# Autodesk Inventor assembly: HTPA22S2M100-K-P4
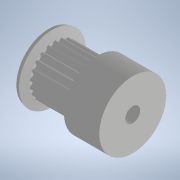
[picture p0: Inventor's stored thumbnail of the model, 180x180]
Saved by Autodesk Inventor 2021 (Build 250183000, 183)
## iProperties
Category: PARTsolutions
Company: MISUMI
Created: 2025-03-04
Part Number: HTPA22S2M100-K-P4
Catalog Web Link: www.cadenas.de
Description: HTPA_ _S2M040, HTPA_ _S2M060, HTPA_ _S2M100, HTPB_ _S2M040, HTPB_ _S2M060, HTPB_ _S2M100, HTPK_ _S2M040, HTPK_ _S2M060, HTPK_ _S2M100, HTPN_ _S2M040, HTPN_ _S2M060, HTPN_ _S2M100, HTPT_ _S2M040, HTPT_ _S2M060, HTPM_ _S2M040, HTPM_ _S2M060, HTPP_ _S2M040, HTPP_ _S2M060, HTPS_ _S2M040, HTPS_ _S2M060, HTPS_ _S2M100-High Torque Timing Pulleys S2M Type
Vendor: MISUMI
Document SubType Name: Assembly
Designer: psAdmin
Manufacturer: MISUMI
Mass: 3.936 g
Surface Area: 24.8143 cm^2
Volume: 3.936 cm^3
Density: 1 g/cm^3
Title: HTPA22S2M100-K-P4
Author: Cadenas PARTsolutions
Comments: High Torque Timing Pulleys S2M Type
PSOL_IDENT_0: {$CADENAS_DATA/23d-libs/misumi/metric/51_timing_pulleys/htpm_s2m_asmtab.prj},744 {VTYP=3D},{STYP=ASS
PSOL_IDENT_1: TAB},{NB=HTPA22S2M100-K-P4},{LINA=HTPA22S2M100-K-P4},{NN=HTPA_ _S2M040, HTPA_ _S2M060, HTPA_ _S2M100
PSOL_IDENT_2: , HTPB_ _S2M040, HTPB_ _S2M060, HTPB_ _S2M100, HTPK_ _S2M040, HTPK_ _S2M060, HTPK_ _S2M100, HTPN_ _S
PSOL_IDENT_3: 2M040, HTPN_ _S2M060, HTPN_ _S2M100, HTPT_ _S2M040, HTPT_ _S2M060, HTPM_ _S2M040, HTPM_ _S2M060, HTP
PSOL_IDENT_4: P_ _S2M040, HTPP_ _S2M060, HTPS_ _S2M040, HTPS_ _S2M060, HTPS_ _S2M100},{DATE=13.01.2023 00:39:47},{
PSOL_IDENT_5: GEOMDATE=09.12.2022 07:33:44},{VERSION=},{LINEID=70},{WBVAR=MATP,ST,TNW,PS,SBS,DD,Z,J,Q,R,S,T,ALT1,A
PSOL_IDENT_6: LT2,M,QSC,QFC,QTC,ALT3,K,KSC,KFC,KTC,ALT4,ZM,ZSC,ZFC,ZTC,ALT5,ALT6,ALT7,FC,ALT8,SRG,ALT9,BTC,TL,ALT1
PSOL_IDENT_7: 0,TPC,ALT11,BC,ALT12,SLH,ALT13,BN},{WBNUMERIC=DD,Z,J,Q,R,S,T,QSC,QFC,QTC,K,KSC,KFC,KTC,ZSC,ZFC,ZTC,F
PSOL_IDENT_8: C,SRG,BTC,TL,BC,SLH,BN}  {NB=HTPA22S2M100-K-P4},{LINA=HTPA22S2M100-K-P4},{KT=DUMMY},{PN=HTPA22S2M100
PSOL_IDENT_9: -K-P4},{TYPE=HTPA},{MATP=A2017},{MATPALG= 'A2017','Aluminum Alloy 2000 series','S45CE','1045 Carbon
PSOL_IDENT_10: Steel Equivalent','SUS304','304 Stainless Steel' },{ST=CA},{STALG= 'CA' , 'Clear Anodize', 'BA','Bla
PSOL_IDENT_11: ck Anodize','HAT','Hard Clear Anodize' , 'ENP' , 'Electroless Nickel Plating' },{NT=22},{TNW=S2M100}
PSOL_IDENT_12: ,{TNWALG= 'S2M040', 'S2M060','S2M100' },{BW=10},{PS=K},{PSALG='A','K'},{SBS=P},{SBSALG='H','Round Ho
PSOL_IDENT_13: le','P','Round Hole + Tap'},{SHSA= 'H', 'Round Hole','V','Stepped Hole','Y','Both Ends Stepped Hole'
PSOL_IDENT_14: ,'WB','Double Stepped Hole' },{SHSB='H','Round Hole','P','Round Hole + Tap','N','New JIS Keywayed Bo
PSOL_IDENT_15: re + Tap (Standard)','NK','New JIS Keywayed Bore + Tap (width 4.0mm, height 1.8mm)','C','Old JIS Key
PSOL_IDENT_16: wayed Bore + Tap','V','Stepped Hole','F','Stepped Hole (Counterbore holes on the boss side)' },{SHSK='
PSOL_IDENT_17: H','Round Hole','P','Round Hole + Tap'},{SBSPN=-P4},{DD=4.00},{DDALG=[3:4/1],4.5,[5:6/1]},{DDHA=[3:4
PSOL_IDENT_18: /1],4.5,[5:6/1],6.35,[7:7/1]},{DDHBK=[3:4/1],4.5,[5:6/1]},{DDPA=0},{DDPBK=[3:4/1],4.5,[5:6/1]},{DDNA=
PSOL_IDENT_19: 0},{DDNBK=0},{DDNK=0},{DDCA=0},{DDCBK=0},{DDVA=0},{DDVF=[3:4/1]},{DDY=[3:5/1]},{DDWB=[3:3/1]},{Z=0},
PSOL_IDENT_20: {ZALG=[0]},{ZQRMIN=6},{ZAMAX=0},{ZBMAX=6},{DDZ=4},{J=0.0},{JALG=[0]},{JMAX=0},{JMIN=2},{JPN=},{QRMAX=
PSOL_IDENT_21: 7},{QRMIN=6},{WBRMAX=-2.00},{WBQMIN=8},{Q=0},{QALG=[0]},{QPN=},{R=0},{RALG=[0]},{S=0.0},{SALG=[0]},{
PSOL_IDENT_22: SPN=},{SMAX=9},{T=0.0},{TALG=[0]},{TPN=},{TMAX=12},{A=11},{W=15},{L=23},{PD=14.01},{OD=13.50},{D=18}
PSOL_IDENT_23: ,{DALG=18},{DE=18},{F=18},{E=11},{BBK=0.000},{TTK=0.0},{TT=1},{WL=23.000},{ALT1=},{ALT1ALG= '','w/o
PSOL_IDENT_24: KC90 (Set Screw Angle)','KC90','with KC90 (Set Screw Angle)' },{ANG=120.000},{ALT1PN=},{ALT2=},{ALT2
PSOL_IDENT_25: ALG= '','Not applicable' },{M=N/A},{MALG= 'N/A' },{MFTALG= 'N/A' },{MSALG= 'N/A' },{M3D=0.000},{KDML=
PSOL_IDENT_26: 0},{ML=0},{MUL=0},{PITCH=0},{QSC=0.0},{QSCALG=0},{QFC=0.0},{QFCALG=0},{QTC=0.0},{QTCALG=0},{QPCDMIN=
PSOL_IDENT_27: 0},{QPCDMINALG=0},{QPCDMAX=14},{ALT2PN=},{ALT3=},{ALT3ALG= '','Not applicable' },{K=0.0},{KALG=0},{K
PSOL_IDENT_28: MIN=4},{KFTMAX=0.0},{KSMAX=0.0},{KSC=0.0},{KSCALG=0},{KFC=0.0},{KFCALG=0},{KTC=0.0},{KTCALG=0},{KPCD
PSOL_IDENT_29: MIN=8},{KPCDMINALG=8},{KPCDMAX=0},{KSCMIN=8.0},{KSCMINALG=8},{ALT3PN=},{ALT4=},{ALT4ALG= '','Not app
PSOL_IDENT_30: licable' },{ALT4MIN=14.5},{ALT4MAX=0.5},{ZM=N/A},{ZMALG= 'N/A' },{ZMSALG= 'N/A' },{ZMFTALG= 'N/A' },
PSOL_IDENT_31: {ZMDD1=0.0},{ZMDD2=0.0},{ZMHH=0.0},{ZSC=0.0},{ZSCALG=[0]},{ZFC=0.0},{ZFCALG=[0]},{ZTC=0.0},{ZTCALG=[
PSOL_IDENT_32: 0]},{ZPCDMIN=0},{ZPCDMINALG=0},{ZPCDMAX=7},{ALT4PN=},{ALT5=},{ALT5ALG= '','Flange Attached','NFC','w
PSOL_IDENT_33: ith NFC (Flange not Attached)' },{ALT5PN=},{ALT6=},{ALT6ALG= '','Not applicable' },{ALT6PN=},{ALT7=}
PSOL_IDENT_34: ,{ALT7ALG= '','w/o FC (Flange Cut)','FC','with FC (Flange Cut)' },{FC=0.0},{FCALG=0},{FCMIN=14.5},{F
PSOL_IDENT_35: CMAX=16.0},{ALT7PN=},{ALT8=},{ALT8ALG= '','Not applicable' },{ALT8ALGALG=14},{ALT8DD2=0},{ALT8MM=0},
PSOL_IDENT_36: {ALT8NN=0},{QC=0},{KC=0},{ZC=0},{SRG=0.0},{SRGALG=[0]},{SRGMAX=0},{DD2=0.0},{MM=0.00},{NN=0.00},{ALT
PSOL_IDENT_37: 8PN=},{ALT9ALG= '','Not applicable' },{ALT9=},{BTC9=6},{TL9=1},{BTC=0},{BTCALG=[0]},{TL=0.0},{TLALG=
PSOL_IDENT_38: [0]},{TLMIN=1.000},{TLMAX=-15.500},{BTCL=0},{BTCD=0},{BTCDALG=11.000},{ALT9PN=},{WLBCTL=23},{ALT10=}
PSOL_IDENT_39: ,{ALT10ALG= '','w/o TPC (Tapped Hole Dimension)','TPC','with TPC (Tapped Hole Dimension)' },{TPC=N/A
PSOL_IDENT_40: },{TPCALG= 'N/A' },{TPCM=3},{ALT10PN=},{ALT11=},{ALT11ALG= '','Not applicable' },{BC=0.0},{BCALG=0},
PSOL_IDENT_41: {BCMIN=6},{BCMAX=7.5},{BCPLANE=18},{M1WBC=18},{ALT11PN=},{ALT12=},{ALT12ALG= '','w/o SLH (Set Screw
PSOL_IDENT_42: Length)','SLH','with SLH (Set Screw Length)' },{SLH=0},{SLHALG=[0]},{ALT12PN=},{ALT13=},{ALT13ALG= ''
PSOL_IDENT_43: , 'Not applicable' },{BN=0.0},{BNALG=0},{BNMIN=8.5},{BNMAX=18},{ALT13PN=},{AC=M3x3},{M1=3},{M1L=3},{
PSOL_IDENT_44: TAP=0.000},{KYY=2},{KTT=7},{PLANE=0},{PPATH=htpm_s2m/htpa_s2m_asmtpl.prj}
NB: HTPA22S2M100-K-P4
NN: 0
NT: 22
NBSYN: $PN.
LINA: HTPA22S2M100-K-P4
CATALOG: Misumi
PN: HTPA22S2M100-K-P4
MATP: Aluminum Alloy 2000 series
ST: Clear Anodize
TNW: S2M100
BW: 10
PS: K
SBS: Round Hole + Tap
DD: 4
Z: 0
J: 0
Q: 0
R: 0
S: 0
T: 0
A: 11
W: 15
L: 23
PD: 14.01
OD: 13.5
D: 18
F: 18
E: 11
TT: 1
ALT1: w/o KC90 (Set Screw Angle)
ALT2: Not applicable
M: N/A
QSC: 0
QFC: 0
QTC: 0
ALT3: Not applicable
K: 0
KSC: 0
KFC: 0
KTC: 0
ALT4: Not applicable
ZM: N/A
ZMDD1: 0
ZMDD2: 0
ZMHH: 0
ZSC: 0
ZFC: 0
ZTC: 0
ALT5: Flange Attached
ALT6: Not applicable
ALT7: w/o FC (Flange Cut)
FC: 0
ALT8: Not applicable
SRG: 0
DD2: 0
MM: 0
ALT9: Not applicable
BTC: 0
TL: 0
BTCL: 0
BTCD: 0
ALT10: w/o TPC (Tapped Hole Dimension)
TPC: N/A
ALT11: Not applicable
BC: 0
ALT12: w/o SLH (Set Screw Length)
SLH: 0
ALT13: Not applicable
BN: 0
AC: M3x3
SUPPLIER: MISUMI
ARTICLENO: HTPA22S2M100-K-P4
BOMINFO: HTPA22S2M100-K-P4
CREATOR: CADENAS GmbH
## Documents named in this file (3)
- e:\temp\worker_COMMON_13\temp\tmp_1524_272_tdsmI\format_0\HTPA22S2M100-K-P4.iam
- e:\temp\worker_COMMON_13\temp\tmp_1524_272_tdsmI\format_0\HTPA22S2M100-K-P4_a.ipt
- e:\temp\worker_COMMON_13\temp\tmp_1524_272_tdsmI\format_0\SET-SCREW3-3.ipt
## Components (3 placed, 2 different names)
1. HTPA22S2M100-K-P4_a:1 — to_s1_Z@1 <-> CP_Z@2, to_s2_Z@1 <-> CP_Z@3
2. SET-SCREW3-3:1 — to_s1_Z@1 <-> CP_Z@2
3. SET-SCREW3-3:2 — to_s2_Z@1 <-> CP_Z@3
## Relationships (2: Mate 2)
- to_s1_Z@1 <-> CP_Z@2 [Mate]: HTPA22S2M100-K-P4_a:1 ↔ SET-SCREW3-3:1
- to_s2_Z@1 <-> CP_Z@3 [Mate]: HTPA22S2M100-K-P4_a:1 ↔ SET-SCREW3-3:2
